# Autodesk Inventor assembly: Chessboard Design
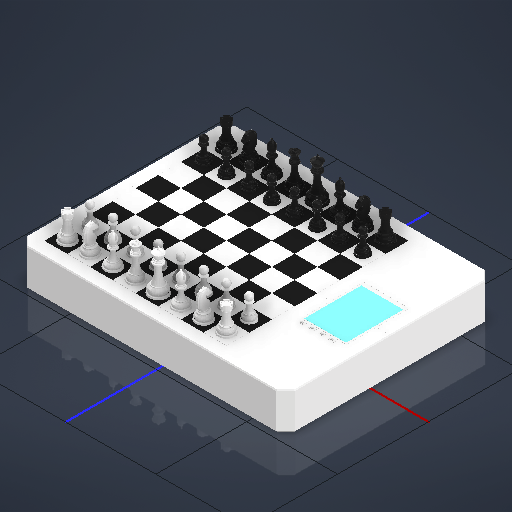
[picture p0: Inventor's stored thumbnail of the model, 512x512]
Saved by Autodesk Inventor 2026 (Build 300175000, 175)
## iProperties
Created: 2025-06-14
Part Number: Chessboard Design
Document SubType Name: Assembly
Designer: ckyiu
Author: ckyiu
## Documents named in this file (3)
- F:\Chessboard-Design\Design\Case\Chessboard Design.iam
- F:\Chessboard-Design\Design\Case\Case.iam
- F:\Chessboard-Design\Design\Core\Chessboard Design Core.iam
## Components (2 placed, 2 different names)
1. Case:1 [sub-assembly] — Insert:1, Insert:2
2. Chessboard Design Core:1 [sub-assembly] — Insert:1, Insert:2
## Relationships (2: Insert 2)
- Insert:1: Case:1 ↔ Chessboard Design Core:1
- Insert:2: Case:1 ↔ Chessboard Design Core:1
